# Autodesk Inventor assembly: Intake new robot
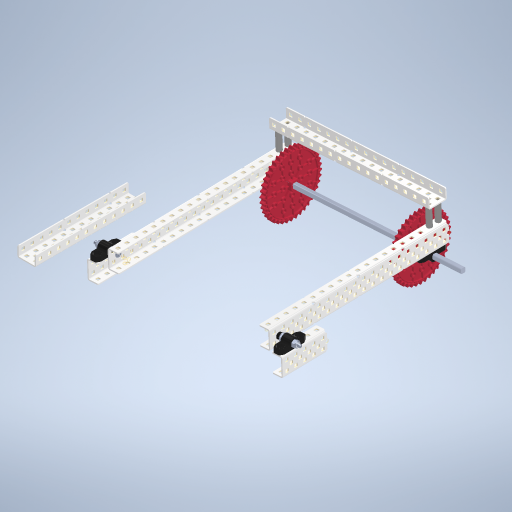
[picture p0: Inventor's stored thumbnail of the model, 512x512]
Saved by Autodesk Inventor 2023 (Build 270158000, 158)
## iProperties
Created: 2023-12-04
Part Number: Intake new robot
Document SubType Name: Assembly
Designer: diego
Author: diego
## Documents named in this file (21)
- C:\Users\Robodox\Documents\GitHub\2024-599Z\Cad\Intake new robot.iam
- C:\Users\Robodox\Documents\GitHub\2024-599Z\Cad\VEX-CAD-Inventor-1.4.0\Structure\C Channel\Aluminum 1x2x1\Alu C 1x2x1x20.ipt
- C:\Users\Robodox\Documents\GitHub\2024-599Z\Cad\VEX-CAD-Inventor-1.4.0\Structure\C Channel\Aluminum 1x2x1\Alu C 1x2x1x5.ipt
- C:\Users\Robodox\Documents\GitHub\2024-599Z\Cad\VEX-CAD-Inventor-1.4.0\Motion\Shaft HS\HS Pillow Bearing Block.ipt
- C:\Users\Robodox\Documents\GitHub\2024-599Z\Cad\VEX-CAD-Inventor-1.4.0\Motion\Spacers\Spacer Plastic\PSpacer 4.6.ipt
- C:\Users\diego\OneDrive\Documents\GitHub\2024-599Z\2024-599Z\Cad\VEX-CAD-Inventor-1.4.0\Motion\Spacers\Spacer Plastic.ipt
- C:\Users\Robodox\Documents\GitHub\2024-599Z\Cad\VEX-CAD-Inventor-1.4.0\Structure\Hardware\Nut Keps.ipt
- C:\Users\Robodox\Documents\GitHub\2024-599Z\Cad\VEX-CAD-Inventor-1.4.0\Structure\Hardware\Screw Steel - Star\SScrew Star Smooth 1.250.ipt
- C:\Users\diego\OneDrive\Documents\GitHub\2024-599Z\2024-599Z\Cad\VEX-CAD-Inventor-1.4.0\Structure\Hardware\Screw Steel - Star.ipt
- C:\Users\Robodox\Documents\GitHub\2024-599Z\Cad\VEX-CAD-Inventor-1.4.0\Structure\C Channel\Aluminum 1x2x1\Alu C 1x2x1x1.ipt
- C:\Users\Robodox\Documents\GitHub\2024-599Z\Cad\VEX-CAD-Inventor-1.4.0\Structure\Hardware\Nut Nylock_CPY_MIR.ipt
- C:\Users\diego\OneDrive\Documents\GitHub\2024-599Z\2024-599Z\Cad\VEX-CAD-Inventor-1.4.0\Motion\Shaft HS\Shaft HS.ipt
- C:\Users\Robodox\Documents\GitHub\2024-599Z\Cad\VEX-CAD-Inventor-1.4.0\Motion\Shaft HS\HS Spacer\HSpacer .0625.ipt
- C:\Users\diego\OneDrive\Documents\GitHub\2024-599Z\2024-599Z\Cad\VEX-CAD-Inventor-1.4.0\Motion\Shaft HS\HS Spacer.ipt
- C:\Users\Robodox\Documents\GitHub\2024-599Z\Cad\VEX-CAD-Inventor-1.4.0\Motion\Sprockets\6P Sprocket\6P 40T Sprocket, No Insert.iam
- C:\Users\diego\OneDrive\Documents\GitHub\2024-599Z\2024-599Z\Cad\VEX-CAD-Inventor-1.4.0\Motion\Sprockets\6P Sprocket.iam
- C:\Users\Robodox\Documents\GitHub\2024-599Z\Cad\VEX-CAD-Inventor-1.4.0\Motion\Shaft HS\Shaft HS\Shaft HS 10.0 in.ipt
- C:\Users\Robodox\Documents\GitHub\2024-599Z\Cad\VEX-CAD-Inventor-1.4.0\Structure\C Channel\Aluminum 1x2x1\Alu C 1x2x1x17.ipt
- C:\Users\Robodox\Documents\GitHub\2024-599Z\Cad\VEX-CAD-Inventor-1.4.0\Structure\Standoff\Standoff 1.00.ipt
- C:\Users\Robodox\Documents\GitHub\2024-599Z\Cad\VEX-CAD-Inventor-1.4.0\Structure\Standoff.ipt
- C:\Users\Robodox\Documents\GitHub\2024-599Z\Cad\VEX-CAD-Inventor-1.4.0\Structure\C Channel\Aluminum 1x2x1\Alu C 1x2x1x12.ipt
## Components (30 placed, 14 different names)
1. Alu C 1x2x1x20:1 — Insert:8, Insert:9, Insert:17, Insert:18, Insert:23, Insert:24
2. Alu C 1x2x1x20:2 — Insert:5, Insert:6, Insert:15, Insert:16, Insert:25, Insert:26
3. Alu C 1x2x1x5:1 — Insert:3, Insert:4
4. Alu C 1x2x1x5:2 — Insert:1, Insert:2
5. HS Pillow Bearing Block:1 — Insert:1, Insert:2, Mate:1, Mate:2
6. HS Pillow Bearing Block:2 — Insert:3, Insert:4, Mate:3, Mate:4
7. PSpacer 4.6:1 — Insert:6, Insert:7
8. PSpacer 4.6:2 — Insert:8, Insert:10
9. Nut Keps:1 — Insert:10
10. Nut Keps:2 — Insert:7
11. SScrew Star Smooth 1.250:1 — Insert:9, Insert:13, Insert:14
12. SScrew Star Smooth 1.250:2 — Insert:5, Insert:11, Insert:12
13. HS Pillow Bearing Block:3 — Insert:17, Insert:18, Mate:16
14. HS Pillow Bearing Block:4 — Insert:15, Insert:16, Mate:11, Mate:14
15. Alu C 1x2x1x1:1 — Insert:13, Mate:3, Mate:4
16. Alu C 1x2x1x1:2 — Insert:11, Mate:1, Mate:2
17. Nut Nylock_CPY_MIR:1 — Insert:12
18. Nut Nylock_CPY_MIR:2 — Insert:14
19. HSpacer .0625:1 — Mate:15, Mate:16
20. HSpacer .0625:2 — Mate:12, Mate:13, Mate:14
21. HSpacer .0625:3 — Mate:11, Insert:20
22. 6P 40T Sprocket, No Insert:1 [sub-assembly]
23. 6P 40T Sprocket, No Insert:2 [sub-assembly] — Insert:20
24. Shaft HS 10.0 in:2 — Mate:12, Mate:13, Mate:15
25. Alu C 1x2x1x17:1 — Insert:27, Insert:28, Insert:29, Mate:17
26. Standoff 1.00:1 — Insert:24, Mate:17
27. Standoff 1.00:2 — Insert:25, Insert:28
28. Standoff 1.00:3 — Insert:23, Insert:29
29. Standoff 1.00:4 — Insert:26, Insert:27
30. Alu C 1x2x1x12:1
## Relationships (37: Insert 26, Mate 11)
- Insert:1: Alu C 1x2x1x5:2 ↔ HS Pillow Bearing Block:1
- Insert:2: Alu C 1x2x1x5:2 ↔ HS Pillow Bearing Block:1
- Insert:3: Alu C 1x2x1x5:1 ↔ HS Pillow Bearing Block:2
- Insert:4: Alu C 1x2x1x5:1 ↔ HS Pillow Bearing Block:2
- Insert:5: Alu C 1x2x1x20:2 ↔ SScrew Star Smooth 1.250:2
- Insert:6: Alu C 1x2x1x20:2 ↔ PSpacer 4.6:1
- Insert:7: PSpacer 4.6:1 ↔ Nut Keps:2
- Insert:8: Alu C 1x2x1x20:1 ↔ PSpacer 4.6:2
- Insert:9: Alu C 1x2x1x20:1 ↔ SScrew Star Smooth 1.250:1
- Insert:10: PSpacer 4.6:2 ↔ Nut Keps:1
- Insert:11 (-47.1932 mm): SScrew Star Smooth 1.250:2 ↔ Alu C 1x2x1x1:2
- Mate:1: HS Pillow Bearing Block:1 ↔ Alu C 1x2x1x1:2
- Mate:2: HS Pillow Bearing Block:1 ↔ Alu C 1x2x1x1:2
- Insert:12 (-9.398 mm): SScrew Star Smooth 1.250:2 ↔ Nut Nylock_CPY_MIR:1
- Insert:13 (-47.1678 mm): SScrew Star Smooth 1.250:1 ↔ Alu C 1x2x1x1:1
- Mate:3: HS Pillow Bearing Block:2 ↔ Alu C 1x2x1x1:1
- Mate:4: HS Pillow Bearing Block:2 ↔ Alu C 1x2x1x1:1
- Insert:14 (-9.398 mm): SScrew Star Smooth 1.250:1 ↔ Nut Nylock_CPY_MIR:2
- Insert:15: Alu C 1x2x1x20:2 ↔ HS Pillow Bearing Block:4
- Insert:16: Alu C 1x2x1x20:2 ↔ HS Pillow Bearing Block:4
- Insert:17: Alu C 1x2x1x20:1 ↔ HS Pillow Bearing Block:3
- Insert:18: Alu C 1x2x1x20:1 ↔ HS Pillow Bearing Block:3
- Mate:11: HS Pillow Bearing Block:4 ↔ HSpacer .0625:3
- Insert:20: HSpacer .0625:3 ↔ 6P 40T Sprocket, No Insert:2
- Mate:12: HSpacer .0625:2 ↔ Shaft HS 10.0 in:2
- Mate:13: HSpacer .0625:2 ↔ Shaft HS 10.0 in:2
- Mate:14: HS Pillow Bearing Block:4 ↔ HSpacer .0625:2
- Mate:15: HSpacer .0625:1 ↔ Shaft HS 10.0 in:2
- Mate:16: HS Pillow Bearing Block:3 ↔ HSpacer .0625:1
- Insert:23: Alu C 1x2x1x20:1 ↔ Standoff 1.00:3
- Insert:24: Alu C 1x2x1x20:1 ↔ Standoff 1.00:1
- Insert:25: Alu C 1x2x1x20:2 ↔ Standoff 1.00:2
- Insert:26: Alu C 1x2x1x20:2 ↔ Standoff 1.00:4
- Insert:27: Alu C 1x2x1x17:1 ↔ Standoff 1.00:4
- Insert:28: Alu C 1x2x1x17:1 ↔ Standoff 1.00:2
- Insert:29: Alu C 1x2x1x17:1 ↔ Standoff 1.00:3
- Mate:17: Alu C 1x2x1x17:1 ↔ Standoff 1.00:1
